# Autodesk Inventor assembly: ASY MSC 0130 cone exit back
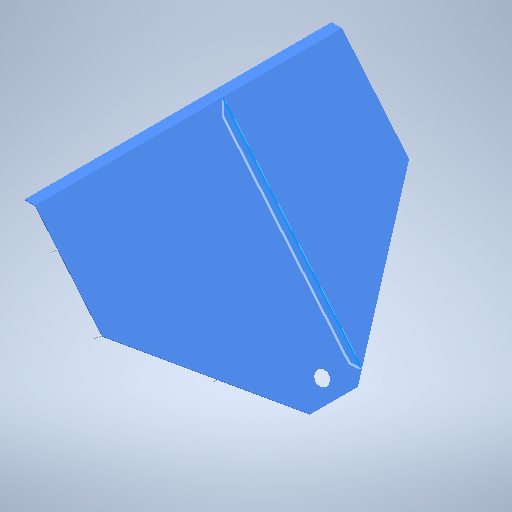
[picture p0: Inventor's stored thumbnail of the model, 512x512]
Saved by Autodesk Inventor 2025 (Build 290162010, 162A)
## iProperties
Created: 2024-08-26
Part Number: ASY MSC 0130 cone exit back
Document SubType Name: Assembly
Designer: pokla
Author: pokla
## Documents named in this file (6)
- C:\Users\pokla\Documents\Inventor\Отстойник осветлитель\Manturovo_Se-clar-Gleb\ASY MSC 0130 cone exit back.iam
- C:\Users\pokla\Documents\Inventor\Отстойник осветлитель\Manturovo_Se-clar-Gleb\конус\MSC 016 cone exit back.ipt
- C:\Users\pokla\Documents\Inventor\Отстойник осветлитель\Manturovo_Se-clar-Gleb\конус\MSC 0161 stringer cone exit back.ipt
- C:\Users\pokla\Documents\Inventor\Отстойник осветлитель\Manturovo_Se-clar-Gleb\конус\MSC 0162 stringer cone exit back.ipt
- C:\Users\pokla\Documents\Inventor\Отстойник осветлитель\Manturovo_Se-clar-Gleb\конус\MSC 0163 rib cone exit back.ipt
- C:\Users\pokla\Documents\Inventor\Отстойник осветлитель\Manturovo_Se-clar-Gleb\конус\MSC 0164 rib cone exit back.ipt
## Components (8 placed, 5 different names)
1. MSC 016 cone exit back.ipt:1 — Mate:2, Mate:4, Mate:5, Flush:1, Mate:6
2. MSC 0161 stringer cone exit back:1 — Mate:2, Mate:3, Mate:4, Rigid:3, Rigid:4
3. MSC 0161 stringer cone exit back:2 — Rigid:3, Rigid:5
4. MSC 0162 stringer cone exit back:1 — Rigid:4
5. MSC 0162 stringer cone exit back:2 — Rigid:5
6. MSC 0163 rib cone exit back:1 — Mate:5, Flush:1, Mate:6, Rigid:6
7. MSC 0163 rib cone exit back:2 — Rigid:6, Rigid:7
8. MSC 0164 rib cone exit back:1 — Rigid:7
## Relationships (11: Mate 5, WeldJoint 5, Flush 1)
- Mate:2: MSC 016 cone exit back.ipt:1 ↔ MSC 0161 stringer cone exit back:1
- Mate:3 (188.5 mm): MSC 0161 stringer cone exit back:1
- Mate:4 (1 mm): MSC 016 cone exit back.ipt:1 ↔ MSC 0161 stringer cone exit back:1
- Rigid:3 [WeldJoint] (377 mm): MSC 0161 stringer cone exit back:1 ↔ MSC 0161 stringer cone exit back:2
- Rigid:4 [WeldJoint] (377 mm): MSC 0161 stringer cone exit back:1 ↔ MSC 0162 stringer cone exit back:1
- Rigid:5 [WeldJoint] (377 mm): MSC 0161 stringer cone exit back:2 ↔ MSC 0162 stringer cone exit back:2
- Mate:5: MSC 016 cone exit back.ipt:1 ↔ MSC 0163 rib cone exit back:1
- Flush:1: MSC 016 cone exit back.ipt:1 ↔ MSC 0163 rib cone exit back:1
- Mate:6 (188.5 mm): MSC 016 cone exit back.ipt:1 ↔ MSC 0163 rib cone exit back:1
- Rigid:6 [WeldJoint] (377 mm): MSC 0163 rib cone exit back:1 ↔ MSC 0163 rib cone exit back:2
- Rigid:7 [WeldJoint] (377 mm): MSC 0163 rib cone exit back:2 ↔ MSC 0164 rib cone exit back:1
